# Autodesk Inventor assembly: PCB Housing (1)
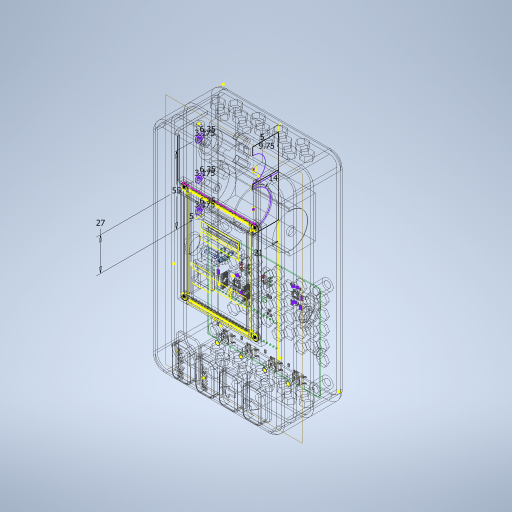
[picture p0: Inventor's stored thumbnail of the model, 512x512]
Saved by Autodesk Inventor 2023 (Build 270158000, 158)
## iProperties
Created: 2024-03-12
Part Number: PCB Housing (1)
Document SubType Name: Assembly
Designer: Pobe Tran
Author: Pobe Tran
## Documents named in this file (13)
- C:\Users\Pobe Tran\OneDrive - McMaster University\YEAR 5\CAPSTONE\PCB Housing (1).iam
- C:\Users\Pobe Tran\OneDrive - McMaster University\YEAR 5\CAPSTONE\Adafruit Screen\2.8TFT Grabcad\Adafruit 2.8TFT.ipt
- C:\Users\Pobe Tran\OneDrive - McMaster University\YEAR 5\CAPSTONE\PCB\PCB1.iam
- C:\Users\Pobe Tran\OneDrive - McMaster University\YEAR 5\CAPSTONE\Pump.ipt
- C:\Users\Pobe Tran\OneDrive - McMaster University\YEAR 5\CAPSTONE\Solenoid Valve.ipt
- C:\Users\Pobe Tran\OneDrive - McMaster University\YEAR 5\CAPSTONE\Bottom Housing.ipt
- C:\Users\Pobe Tran\OneDrive - McMaster University\YEAR 5\CAPSTONE\Valve Tube.ipt
- C:\Users\Pobe Tran\OneDrive - McMaster University\YEAR 5\CAPSTONE\Top Housing.ipt
- C:\Users\Pobe Tran\OneDrive - McMaster University\YEAR 5\CAPSTONE\Lid Cover.ipt
- C:\Users\Pobe Tran\OneDrive - McMaster University\YEAR 5\CAPSTONE\Button - ONOFF.ipt
- C:\Users\Pobe Tran\OneDrive - McMaster University\YEAR 5\CAPSTONE\Button - START.ipt
- C:\Users\Pobe Tran\OneDrive - McMaster University\YEAR 5\CAPSTONE\Button - UP.ipt
- C:\Users\Pobe Tran\OneDrive - McMaster University\YEAR 5\CAPSTONE\Button - DOWN.ipt
## Components (13 placed, 12 different names)
1. Adafruit 2.8TFT:1
2. PCB1:1 [sub-assembly] — Flush:1, Flush:2, Flush:3, Mate:1, Mate:2, Mate:8, Mate:17, Mate:18, Mate:19, Mate:20, Mate:21, Mate:22, Mate:23, Mate:24
3. Pump:1 — Mate:26, Mate:27
4. Bottom Housing:1 — Mate:1, Mate:2, Mate:8, Flush:8, Flush:13, Flush:16, Angle:1, Mate:26, Angle:2, Mate:28
5. Valve Tube:1 — Angle:1, Mate:27
6. Top Housing:1 — Flush:8, Flush:13, Mate:12, Mate:13, Mate:14, Flush:16, Mate:15, Flush:17, Flush:18, Mate:16, Flush:19
7. Adafruit 2.8TFT:2 — Mate:12, Mate:13, Mate:14, Flush:19
8. Lid Cover:1 — Mate:15, Flush:17, Flush:18, Mate:16
9. Button - ONOFF:1 — Mate:17, Mate:18
10. Button - START:1 — Mate:19, Mate:20
11. Button - UP:1 — Mate:21, Mate:22
12. Button - DOWN:1 — Mate:23, Mate:24
13. Solenoid Valve:1 — Angle:2, Mate:28
## Relationships (30: Mate 19, Flush 9, Angle 2)
- Flush:1: PCB1:1
- Flush:2: PCB1:1
- Flush:3: PCB1:1
- Mate:1: PCB1:1 ↔ Bottom Housing:1
- Mate:2: PCB1:1 ↔ Bottom Housing:1
- Mate:8: PCB1:1 ↔ Bottom Housing:1
- Flush:8: Bottom Housing:1 ↔ Top Housing:1
- Flush:13: Bottom Housing:1 ↔ Top Housing:1
- Mate:12: Top Housing:1 ↔ Adafruit 2.8TFT:2
- Mate:13 (0.5 mm): Top Housing:1 ↔ Adafruit 2.8TFT:2
- Mate:14 (0.5 mm): Top Housing:1 ↔ Adafruit 2.8TFT:2
- Flush:16: Bottom Housing:1 ↔ Top Housing:1
- Mate:15: Top Housing:1 ↔ Lid Cover:1
- Flush:17: Top Housing:1 ↔ Lid Cover:1
- Flush:18: Top Housing:1 ↔ Lid Cover:1
- Mate:16: Top Housing:1 ↔ Lid Cover:1
- Mate:17: PCB1:1 ↔ Button - ONOFF:1
- Mate:18: PCB1:1 ↔ Button - ONOFF:1
- Mate:19: PCB1:1 ↔ Button - START:1
- Mate:20: PCB1:1 ↔ Button - START:1
- Mate:21: PCB1:1 ↔ Button - UP:1
- Mate:22: PCB1:1 ↔ Button - UP:1
- Mate:23: PCB1:1 ↔ Button - DOWN:1
- Mate:24: PCB1:1 ↔ Button - DOWN:1
- Flush:19: Top Housing:1 ↔ Adafruit 2.8TFT:2
- Angle:1 (0 deg): Bottom Housing:1 ↔ Valve Tube:1
- Mate:26: Pump:1 ↔ Bottom Housing:1
- Mate:27: Pump:1 ↔ Valve Tube:1
- Angle:2 (45 deg): Bottom Housing:1 ↔ Solenoid Valve:1
- Mate:28: Bottom Housing:1 ↔ Solenoid Valve:1
